# Autodesk Inventor assembly: FEM-Träger-Baugruppe4
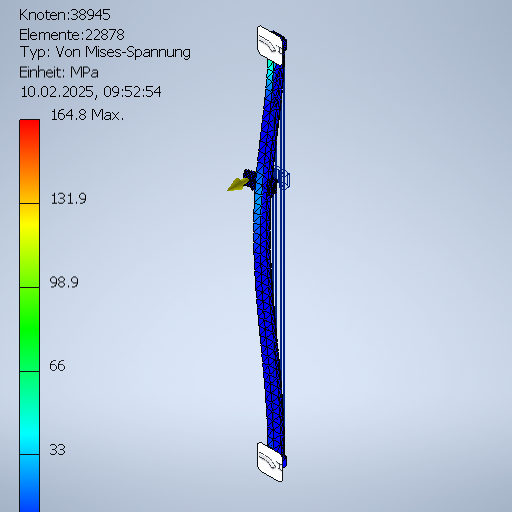
[picture p0: Inventor's stored thumbnail of the model, 512x512]
Saved by Autodesk Inventor 2025 (Build 290162010, 162A)
## iProperties
Created: 2025-02-05
Part Number: FEM-Träger-Baugruppe4
Document SubType Name: Assembly
Designer: Admin
Mass: 496.826 g
Surface Area: 1700.01 cm^2
Volume: 184.01 cm^3
Density: 2.7 g/cm^3
Author: Admin
## Documents named in this file (9)
- C:\Users\Admin\GIT\HDVKBM\CAD\Krandemonstrator\FEM-Träger-Baugruppe8.iam
- C:\Users\Admin\GIT\HDVKBM\CAD\Krandemonstrator\KatzeFEM.ipt
- C:\Users\Admin\GIT\HDVKBM\CAD\Krandemonstrator\TrägerUI - Kopie.ipt
- C:\Users\Admin\GIT\HDVKBM\CAD\Krandemonstrator\FEM-Träger-Baugruppe8\AIP\FEA\eywcr0k68.fins
- C:\Users\Admin\GIT\HDVKBM\CAD\Krandemonstrator\FEM-Träger-Baugruppe8\AIP\FEA\eywcr0k68.fsat
- C:\Users\Admin\GIT\HDVKBM\CAD\Krandemonstrator\FEM-Träger-Baugruppe8\AIP\FEA\eywcr0k68.ftes
- C:\Users\Admin\GIT\HDVKBM\CAD\Krandemonstrator\FEM-Träger-Baugruppe8\AIP\FEA\eywcr0k68.fwiz
- C:\Users\Admin\GIT\HDVKBM\CAD\Krandemonstrator\FEM-Träger-Baugruppe8\AIP\FEA\eywcr0k8w.fmsh
- C:\Users\Admin\GIT\HDVKBM\CAD\Krandemonstrator\FEM-Träger-Baugruppe8\AIP\FEA\eywcr0k8x.fres
## Components (2 placed, 2 different names)
1. TrägerUI - Kopie:1 — Verschiebbar:1
2. KatzeFEM:1 — Verschiebbar:1
## Relationships (1: TranslationJoint 1)
- Verschiebbar:1 [TranslationJoint] (1 mm): TrägerUI - Kopie:1 ↔ KatzeFEM:1
## Named parameters: sa_0 = 50000
note: some values were not read from the file. Shown as the stored number, unit unknown: "sa_0".
